# Autodesk Inventor assembly: Gimble_stand_v2
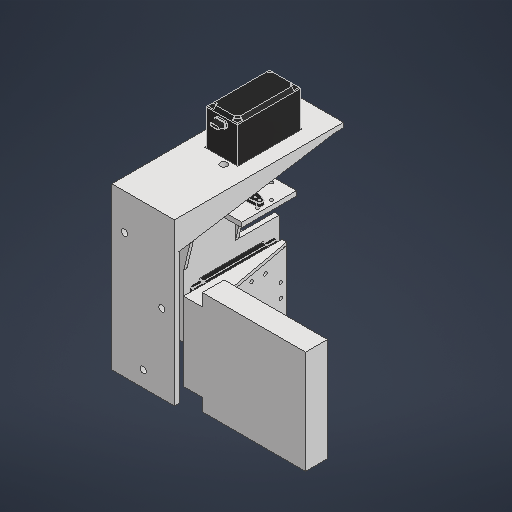
[picture p0: Inventor's stored thumbnail of the model, 512x512]
Saved by Autodesk Inventor 2026 (Build 300175000, 175)
## iProperties
Created: 2025-07-02
Part Number: Gimble_stand_v2
Document SubType Name: Assembly
Designer: user
Author: user
## Documents named in this file (6)
- C:\Users\user\OneDrive - Ashesi University\third_year\System Engineering\Project\ping_pong_mechanism\Gimble_stand_v2.iam
- C:\Users\user\OneDrive - Ashesi University\third_year\System Engineering\Project\ping_pong_mechanism\pan_base_holder_first.ipt
- C:\Users\user\OneDrive - Ashesi University\third_year\System Engineering\Project\ping_pong_mechanism\Servo Futaba S3003 v6\Servo Futaba S3003 v6\Part4.ipt
- C:\Users\user\OneDrive - Ashesi University\third_year\System Engineering\Project\ping_pong_mechanism\Servo Futaba S3003 v6\Servo Futaba S3003 v6\Aspa_creu_Axix holder_v2_one_flap.ipt
- C:\Users\user\OneDrive - Ashesi University\third_year\System Engineering\Project\ping_pong_mechanism\pan_base_holder_second.ipt
- C:\Users\user\OneDrive - Ashesi University\third_year\System Engineering\Project\ping_pong_mechanism\pan_base_holder_third.ipt
## Components (7 placed, 5 different names)
1. pan_base_holder_first:1 — Mate:1, Mate:2, Mate:3, Flush:1, Mate:7, Mate:14
2. Part4:1 — Mate:1, Mate:2, Mate:3, Mate:4, Mate:5
3. Aspa_creu_Axix holder_v2_one_flap:1 — Mate:4, Mate:5, Mate:6
4. pan_base_holder_second:1 — Mate:6, Flush:1, Mate:7, Mate:8, Mate:9, Mate:10
5. Part4:2 — Mate:8, Mate:9, Mate:10, Mate:11, Mate:12
6. Aspa_creu_Axix holder_v2_one_flap:2 — Mate:11, Mate:12, Mate:13
7. pan_base_holder_third:1 — Mate:13, Mate:14
## Relationships (15: Mate 14, Flush 1)
- Mate:1: pan_base_holder_first:1 ↔ Part4:1
- Mate:2 (0.5 mm): pan_base_holder_first:1 ↔ Part4:1
- Mate:3 (0.25 mm): pan_base_holder_first:1 ↔ Part4:1
- Mate:4: Part4:1 ↔ Aspa_creu_Axix holder_v2_one_flap:1
- Mate:5: Part4:1 ↔ Aspa_creu_Axix holder_v2_one_flap:1
- Mate:6: Aspa_creu_Axix holder_v2_one_flap:1 ↔ pan_base_holder_second:1
- Flush:1: pan_base_holder_first:1 ↔ pan_base_holder_second:1
- Mate:7 (40 mm): pan_base_holder_first:1 ↔ pan_base_holder_second:1
- Mate:8: pan_base_holder_second:1 ↔ Part4:2
- Mate:9 (0.5 mm): pan_base_holder_second:1 ↔ Part4:2
- Mate:10 (0.25 mm): pan_base_holder_second:1 ↔ Part4:2
- Mate:11: Part4:2 ↔ Aspa_creu_Axix holder_v2_one_flap:2
- Mate:12: Part4:2 ↔ Aspa_creu_Axix holder_v2_one_flap:2
- Mate:13: Aspa_creu_Axix holder_v2_one_flap:2 ↔ pan_base_holder_third:1
- Mate:14 (20 mm): pan_base_holder_first:1 ↔ pan_base_holder_third:1
